# Autodesk Inventor assembly: Lamp
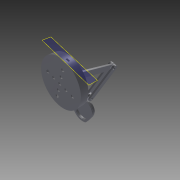
[picture p0: Inventor's stored thumbnail of the model, 180x180]
Saved by Autodesk Inventor 2015 (Build 190159000, 159)
## iProperties
Created: 2017-04-18
Part Number: Lamp
Document SubType Name: Assembly
Designer: Silas
Author: Silas
## Documents named in this file (7)
- D:\Skole\Viborg Tekniske Gymnasium - 2.G\Teknologi\Eksamensprojekt\Lamp.iam
- D:\Skole\Viborg Tekniske Gymnasium - 2.G\Teknologi\Eksamensprojekt\Base top.ipt
- D:\Skole\Viborg Tekniske Gymnasium - 2.G\Teknologi\Eksamensprojekt\Lamp arm 1.ipt
- D:\Skole\Viborg Tekniske Gymnasium - 2.G\Teknologi\Eksamensprojekt\slutskive.ipt
- D:\Skole\Viborg Tekniske Gymnasium - 2.G\Teknologi\Eksamensprojekt\Lamp arm 2.ipt
- D:\Skole\Viborg Tekniske Gymnasium - 2.G\Teknologi\Eksamensprojekt\base bund.ipt
- D:\Skole\Viborg Tekniske Gymnasium - 2.G\Teknologi\Eksamensprojekt\lamp head rev 2.ipt
## Components (12 placed, 6 different names)
1. Base top:1 — Insert:3, Insert:13, Insert:14
2. Lamp arm 1:1 — Insert:1, Insert:2, Insert:4, Insert:5
3. slutskive:1 — Insert:2
4. slutskive:2 — Insert:1, Insert:3
5. slutskive:3 — Insert:5, Insert:7
6. slutskive:4 — Insert:4, Insert:6
7. Lamp arm 2:1 — Insert:6, Insert:12
8. Lamp arm 2:2 — Insert:7, Insert:10
9. slutskive:5 — Insert:10, Insert:15
10. slutskive:6 — Insert:12, Insert:16
11. base bund:1 — Insert:13, Insert:14, Mate:1
12. lamp head rev 2:1 — Insert:15, Insert:16
## Relationships (14: Insert 13, Mate 1)
- Insert:1: Lamp arm 1:1 ↔ slutskive:2
- Insert:2: Lamp arm 1:1 ↔ slutskive:1
- Insert:3: Base top:1 ↔ slutskive:2
- Insert:4: Lamp arm 1:1 ↔ slutskive:4
- Insert:5: Lamp arm 1:1 ↔ slutskive:3
- Insert:6: slutskive:4 ↔ Lamp arm 2:1
- Insert:7: slutskive:3 ↔ Lamp arm 2:2
- Insert:10: Lamp arm 2:2 ↔ slutskive:5
- Insert:12: Lamp arm 2:1 ↔ slutskive:6
- Insert:13: Base top:1 ↔ base bund:1
- Insert:14: Base top:1 ↔ base bund:1
- Mate:1: base bund:1
- Insert:15: slutskive:5 ↔ lamp head rev 2:1
- Insert:16: slutskive:6 ↔ lamp head rev 2:1
